# Autodesk Inventor assembly: リンク_6_1
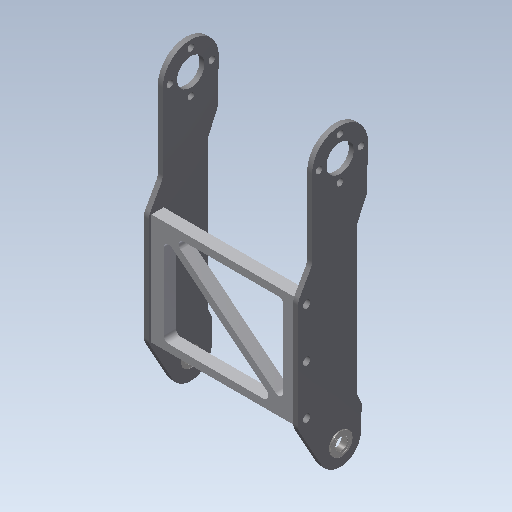
[picture p0: Inventor's stored thumbnail of the model, 512x512]
Saved by Autodesk Inventor 2020 (Build 240168000, 168)
## iProperties
Created: 2016-08-23
Part Number: リンク_6_1
Material: 一般
Document SubType Name: Assembly
Designer: hiro
Mass: 33.7033 g
Surface Area: 186.768 cm^2
Volume: 15.6793 cm^3
Density: 2.14953 g/cm^3
Author: hiro
## Documents named in this file (4)
- C:\Inventor\OpenPlatform_ver3_0\下半身_160823\リンク\リンク_6_4.iam
- C:\Inventor\OpenPlatform_ver3_0\下半身\リンク\ふくらはぎ\リンク_ふくらはぎ_サブフレーム_1_1(予備案).ipt
- C:\Inventor\OpenPlatform_ver3_0\既製品\NSK_RB_MF85ZZ\MF85ZZ.iam
- C:\Inventor\OpenPlatform_ver3_0\下半身_160823\リンク\リンク_メインフレーム_6_2.ipt
## Components (5 placed, 3 different names)
1. リンク_ふくらはぎ_サブフレーム_1_1(予備案):1 — 挿入:25, 挿入:26, 挿入:27, 挿入:32, 挿入:33, 挿入:34
2. MF85ZZ:3 [sub-assembly] — 挿入:31
3. MF85ZZ:4 [sub-assembly] — 挿入:35
4. リンク_メインフレーム_6_2:1 — 挿入:25, 挿入:26, 挿入:27, 挿入:35
5. リンク_メインフレーム_6_2:2 — 挿入:31, 挿入:32, 挿入:33, 挿入:34
## Relationships (8: Insert 8)
- 挿入:25 [Insert]: リンク_ふくらはぎ_サブフレーム_1_1(予備案):1 ↔ リンク_メインフレーム_6_2:1
- 挿入:26 [Insert]: リンク_ふくらはぎ_サブフレーム_1_1(予備案):1 ↔ リンク_メインフレーム_6_2:1
- 挿入:27 [Insert]: リンク_ふくらはぎ_サブフレーム_1_1(予備案):1 ↔ リンク_メインフレーム_6_2:1
- 挿入:31 [Insert]: MF85ZZ:3 ↔ リンク_メインフレーム_6_2:2
- 挿入:32 [Insert]: リンク_ふくらはぎ_サブフレーム_1_1(予備案):1 ↔ リンク_メインフレーム_6_2:2
- 挿入:33 [Insert]: リンク_ふくらはぎ_サブフレーム_1_1(予備案):1 ↔ リンク_メインフレーム_6_2:2
- 挿入:34 [Insert]: リンク_ふくらはぎ_サブフレーム_1_1(予備案):1 ↔ リンク_メインフレーム_6_2:2
- 挿入:35 [Insert]: MF85ZZ:4 ↔ リンク_メインフレーム_6_2:1
